# Autodesk Inventor assembly: nc_nhk14
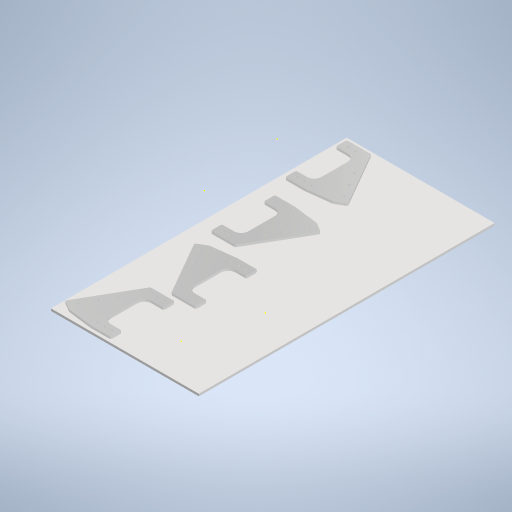
[picture p0: Inventor's stored thumbnail of the model, 512x512]
Saved by Autodesk Inventor 2023 (Build 270158000, 158)
## iProperties
Created: 2022-04-23
Part Number: nc_nhk14
Document SubType Name: Assembly
Designer: yuta
Author: yuta
## Documents named in this file (3)
- C:\Users\yuta\Documents\NHK\nc_nhk14.iam
- C:\Users\yuta\Documents\NHK\NC.port.ipt
- C:\Users\yuta\Downloads\オムニホイール\オムニホイール\ホイールユニット_側板1.ipt
## Components (5 placed, 2 different names)
1. NC.port:1 — メイト:1, フラッシュ:1, メイト:2, メイト:3, メイト:4, メイト:5, フラッシュ:2, フラッシュ:3
2. ホイールユニット_側板1:2 — メイト:1, フラッシュ:1, メイト:2
3. ホイールユニット_側板1:5 — メイト:3
4. ホイールユニット_側板1:7 — メイト:5, フラッシュ:2, フラッシュ:3
5. ホイールユニット_側板1:8 — メイト:4
## Relationships (8: Mate 5, Flush 3)
- メイト:1 [Mate]: NC.port:1 ↔ ホイールユニット_側板1:2
- フラッシュ:1 [Flush] (4 mm): NC.port:1 ↔ ホイールユニット_側板1:2
- メイト:2 [Mate] (-6 mm): NC.port:1 ↔ ホイールユニット_側板1:2
- メイト:3 [Mate]: NC.port:1 ↔ ホイールユニット_側板1:5
- メイト:4 [Mate]: NC.port:1 ↔ ホイールユニット_側板1:8
- メイト:5 [Mate]: NC.port:1 ↔ ホイールユニット_側板1:7
- フラッシュ:2 [Flush] (6 mm): NC.port:1 ↔ ホイールユニット_側板1:7
- フラッシュ:3 [Flush] (6 mm): NC.port:1 ↔ ホイールユニット_側板1:7
